# Autodesk Inventor assembly: Assembly_Lambda_2_rotator
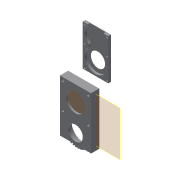
[picture p0: Inventor's stored thumbnail of the model, 180x180]
Saved by Autodesk Inventor 2019 (Build 230136000, 136)
## iProperties
Created: 2019-07-08
Part Number: Assembly_Lambda_2_rotator
Document SubType Name: Assembly
Designer: diederichbenedict
Author: diederichbenedict
## Documents named in this file (6)
- C:\Users\diederichbenedict\Dropbox\Dokumente\Promotion\PROJECTS\STORMoChip\INVENTOR\Nanoscopy-on-a-cheap\LambdaHalfPlateRotator\Assembly_LambdaHalfPlate_rotator.iam
- C:\Users\diederichbenedict\Dropbox\Dokumente\Promotion\PROJECTS\STORMoChip\INVENTOR\Nanoscopy-on-a-cheap\00_Lambda_2_Plate.ipt
- C:\Users\diederichbenedict\Dropbox\Dokumente\Promotion\PROJECTS\STORMoChip\INVENTOR\Nanoscopy-on-a-cheap\200_Holder_Lambdaplate_1.ipt
- C:\Users\diederichbenedict\Dropbox\Dokumente\Promotion\PROJECTS\STORMoChip\INVENTOR\Nanoscopy-on-a-cheap\200_Gearbox.ipt
- C:\Users\diederichbenedict\Dropbox\Dokumente\Promotion\PROJECTS\STORMoChip\INVENTOR\Nanoscopy-on-a-cheap\200_Lambdaplatte_2_conterplate.ipt
- C:\Users\diederichbenedict\Dropbox\Dokumente\Promotion\PROJECTS\STORMoChip\INVENTOR\Nanoscopy-on-a-cheap\200_Gearbox_conterplate.ipt
## Components (6 placed, 5 different names)
1. 00_Lambda_2_Plate:1 — Insert:1, Flush:1
2. 200_Lambdaplatte_2_conterplate:1
3. 200_Gearbox_conterplate:1 — Flush:1, Insert:2
4. 200_Gearbox:1
5. 200_Holder_Lambdaplate_1:1 — Insert:1
6. 200_Holder_Lambdaplate_1:2 — Insert:2
## Relationships (3: Insert 2, Flush 1)
- Insert:1: 00_Lambda_2_Plate:1 ↔ 200_Holder_Lambdaplate_1:1
- Flush:1: 00_Lambda_2_Plate:1 ↔ 200_Gearbox_conterplate:1
- Insert:2: 200_Gearbox_conterplate:1 ↔ 200_Holder_Lambdaplate_1:2
